# Autodesk Inventor assembly: Lady Brown
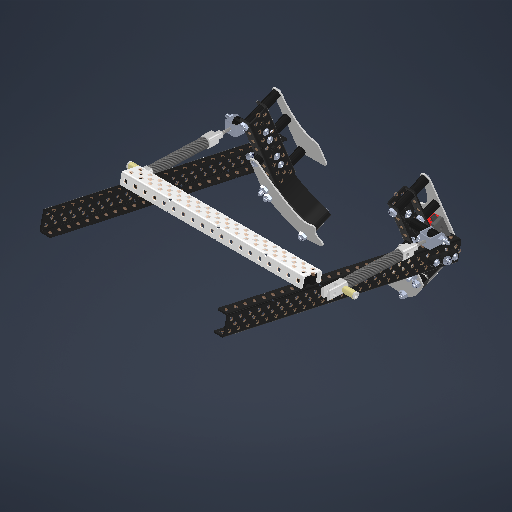
[picture p0: Inventor's stored thumbnail of the model, 512x512]
Saved by Autodesk Inventor 2025 (Build 290162000, 162)
## iProperties
Created: 2024-12-19
Part Number: Lady Brown
Document SubType Name: Assembly
Designer: Juan
Author: Juan
## Documents named in this file (33)
- C:\Users\Juan\Documents\GitHub\ATUM-VRC-High-Stakes-CAD\Robot\Subassemblies\Lady Brown.iam
- C:\Users\Juan\Documents\GitHub\ATUM-VRC-High-Stakes-CAD\VEX-CAD-Inventor\Structure\C Channel\Aluminum 1x2x1\Alu C 1x2x1x25.ipt
- C:\Users\Juan\Documents\GitHub\ATUM-VRC-High-Stakes-CAD\VEX-CAD-Inventor\Structure\C Channel\Aluminum 1x2x1\Alu C 1x2x1x19.ipt
- C:\Users\Juan\Documents\GitHub\ATUM-VRC-High-Stakes-CAD\VEX-CAD-Inventor\Motion\Spacers\Spacer Nylon .375 OD\NSpacer .375 OD x .500.ipt
- C:\Users\Juan\Documents\GitHub\ATUM-VRC-High-Stakes-CAD\VEX-CAD-Inventor\Motion\Spacers\Spacer Nylon .375 OD.ipt
- C:\Users\Juan\Documents\GitHub\ATUM-VRC-High-Stakes-CAD\VEX-CAD-Inventor\Motion\Pneumatics\Reference Parts\Pistons\Double Acting Piston Body.ipt
- C:\Users\Juan\Documents\GitHub\ATUM-VRC-High-Stakes-CAD\VEX-CAD-Inventor\Motion\Pneumatics\Reference Parts\Pistons\Double Acting Piston Rod.ipt
- C:\Users\Juan\Documents\GitHub\ATUM-VRC-High-Stakes-CAD\VEX-CAD-Inventor\Motion\Pneumatics\Legacy - SMC Pneumatics\Fitting for Cylinders.ipt
- C:\Users\Juan\Documents\GitHub\ATUM-VRC-High-Stakes-CAD\VEX-CAD-Inventor\Motion\Shaft LS\Bearing Flat.ipt
- C:\Users\Juan\Documents\GitHub\ATUM-VRC-High-Stakes-CAD\VEX-CAD-Inventor\Structure\Hardware\Screw Steel - Star\SScrew Star Smooth .500.ipt
- C:\Users\Juan\Documents\GitHub\ATUM-VRC-High-Stakes-CAD\VEX-CAD-Inventor\Structure\Hardware\Screw Steel - Star.ipt
- C:\Users\Juan\Documents\GitHub\ATUM-VRC-High-Stakes-CAD\VEX-CAD-Inventor\Structure\C Channel\Aluminum 1x3x1\Alu C 1x3x1x11.ipt
- C:\Users\Juan\Documents\GitHub\ATUM-VRC-High-Stakes-CAD\VEX-CAD-Inventor\Motion\1-Post Bearing Flat Hex Retainer.ipt
- C:\Users\Juan\Documents\GitHub\ATUM-VRC-High-Stakes-CAD\VEX-CAD-Inventor\Motion\Pneumatics\Legacy - SMC Pneumatics\Cylinder Mount.ipt
- C:\Users\Juan\Documents\GitHub\ATUM-VRC-High-Stakes-CAD\VEX-CAD-Inventor\Motion\Spacers\Spacer Nylon .375 OD\NSpacer .375 OD x .375.ipt
- C:\Users\Juan\Documents\GitHub\ATUM-VRC-High-Stakes-CAD\VEX-CAD-Inventor\Structure\Hardware\Screw Steel - Star\SScrew Star Smooth 2.250.ipt
- C:\Users\Juan\Documents\GitHub\ATUM-VRC-High-Stakes-CAD\VEX-CAD-Inventor\Structure\Hardware\Nut Nylock.ipt
- C:\Users\Juan\Documents\GitHub\ATUM-VRC-High-Stakes-CAD\VEX-CAD-Inventor\Structure\Hardware\Screw Steel - Star\SScrew Star Smooth 1.750.ipt
- C:\Users\Juan\Documents\GitHub\ATUM-VRC-High-Stakes-CAD\VEX-CAD-Inventor\Structure\Hardware\Nut Thin Nylock.ipt
- C:\Users\Juan\Documents\GitHub\ATUM-VRC-High-Stakes-CAD\VEX-CAD-Inventor\Structure\Hardware\Screw Steel - Star\SScrew Star Smooth .375.ipt
- C:\Users\Juan\Documents\GitHub\ATUM-VRC-High-Stakes-CAD\VEX-CAD-Inventor\Motion\Spacers\Spacer Nylon .375 OD\NSpacer .375 OD x .250.ipt
- C:\Users\Juan\Documents\GitHub\ATUM-VRC-High-Stakes-CAD\Protobot\Lady Brown Tabs.ipt
- C:\Users\Juan\Documents\GitHub\ATUM-VRC-High-Stakes-CAD\Protobot\Lady Brown Tab Top.ipt
- C:\Users\Juan\Documents\GitHub\ATUM-VRC-High-Stakes-CAD\VEX-CAD-Inventor\Structure\C Channel\Aluminum 1x2x1\Alu C 1x2x1x8.ipt
- C:\Users\Juan\Documents\GitHub\ATUM-VRC-High-Stakes-CAD\VEX-CAD-Inventor\Electronics\Sensors\Line Tracker - V2.ipt
- C:\Users\Juan\Documents\GitHub\ATUM-VRC-High-Stakes-CAD\Protobot\Lady Brown Ring Stop.ipt
- C:\Users\Juan\Documents\GitHub\ATUM-VRC-High-Stakes-CAD\VEX-CAD-Inventor\Motion\Spacers\Washer Steel\SWasher .375 OD x .062500.ipt
- C:\Users\Juan\Documents\GitHub\ATUM-VRC-High-Stakes-CAD\VEX-CAD-Inventor\Motion\Spacers\Washer Steel.ipt
- C:\Users\Juan\Documents\GitHub\ATUM-VRC-High-Stakes-CAD\VEX-CAD-Inventor\Structure\Hardware\Screw Steel - Star\SScrew Star Smooth 1.500.ipt
- C:\Users\Juan\Documents\GitHub\ATUM-VRC-High-Stakes-CAD\VEX-CAD-Inventor\Structure\Hardware\Screw Steel - Star\SScrew Star Smooth 2.000.ipt
- C:\Users\Juan\Documents\GitHub\ATUM-VRC-High-Stakes-CAD\VEX-CAD-Inventor\Structure\Hardware\Screw Steel - Star\SScrew Star Smooth 2.500.ipt
- C:\Users\Juan\Documents\GitHub\ATUM-VRC-High-Stakes-CAD\VEX-CAD-Inventor\Structure\Hardware\Screw Steel - Star\SScrew Star Smooth 1.250.ipt
- C:\Users\Juan\Documents\GitHub\ATUM-VRC-High-Stakes-CAD\VEX-CAD-Inventor\Structure\Hardware\Screw Steel - Star\SScrew Star Smooth .625.ipt
## Components (118 placed, 29 different names)
1. Alu C 1x2x1x25:1
2. Alu C 1x2x1x25:2
3. Alu C 1x2x1x19:1
4. NSpacer .375 OD x .500:1
5. NSpacer .375 OD x .500:2
6. Double Acting Piston Body:1
7. Double Acting Piston Rod:1
8. Fitting for Cylinders:1
9. Bearing Flat:1
10. SScrew Star Smooth .500:1
11. SScrew Star Smooth .500:2
12. Alu C 1x3x1x11:1
13. 1-Post Bearing Flat Hex Retainer:1
14. 1-Post Bearing Flat Hex Retainer:2 — Mate:77
15. Cylinder Mount:1
16. NSpacer .375 OD x .375:3 — Mate:78
17. NSpacer .375 OD x .500:4 — Mate:79
18. NSpacer .375 OD x .375:5
19. NSpacer .375 OD x .500:6
20. SScrew Star Smooth 2.250:3
21. Nut Nylock:1
22. SScrew Star Smooth 1.750:4
23. Nut Thin Nylock:1
24. Nut Nylock:2
25. SScrew Star Smooth .375:5
26. SScrew Star Smooth .375:6
27. Nut Nylock:3
28. Double Acting Piston Body:2
29. Double Acting Piston Rod:2
30. NSpacer .375 OD x .500:13
31. NSpacer .375 OD x .375:14
32. Nut Thin Nylock:4
33. Nut Thin Nylock:3
34. Nut Thin Nylock:6
35. Nut Thin Nylock:5
36. SScrew Star Smooth 2.250:12
37. NSpacer .375 OD x .500:12
38. Fitting for Cylinders:2
39. Bearing Flat:2
40. SScrew Star Smooth .500:7
41. SScrew Star Smooth .500:8
42. Alu C 1x3x1x11:2
43. NSpacer .375 OD x .500:10
44. NSpacer .375 OD x .500:11
45. Cylinder Mount:2
46. NSpacer .375 OD x .500:7
47. Nut Nylock:4
48. Nut Thin Nylock:2
49. Nut Nylock:5
50. SScrew Star Smooth .375:9
51. SScrew Star Smooth .375:10
52. Nut Nylock:6
53. 1-Post Bearing Flat Hex Retainer:3 — Mate:93
54. 1-Post Bearing Flat Hex Retainer:4 — Mate:94
55. SScrew Star Smooth 1.750:11
56. NSpacer .375 OD x .500:8 — Mate:95
57. NSpacer .375 OD x .375:9
58. NSpacer .375 OD x .375:15 — Rigid:36, Rigid:41
59. NSpacer .375 OD x .375:16 — Rigid:36, Mate:73, Mate:75, Mate:76
60. NSpacer .375 OD x .250:17 — Mate:70, Mate:72, Rigid:42
61. NSpacer .375 OD x .250:18 — Mate:71, Rigid:43
62. Lady Brown Tabs:2 — Mate:70, Mate:71, Mate:72, Mate:88, Rigid:54, Rigid:56, Rigid:67, Rigid:68, Rigid:78, Rigid:83
63. Lady Brown Tab Top:1 — Mate:73, Mate:75, Mate:76, Mate:83, Rigid:72, Rigid:76, Rigid:79
64. NSpacer .375 OD x .375:21 — Rigid:40
65. NSpacer .375 OD x .375:22 — Mate:83
66. Alu C 1x2x1x8:1 — Mate:77, Mate:78, Mate:79, Rigid:40, Rigid:41, Rigid:42, Rigid:43, Flush:1, Mate:84, Mate:85, Rigid:45, Mate:86, Mate:87, Rigid:71, Rigid:74, Rigid:81, Rigid:84
67. Line Tracker - V2:2 — Flush:1, Mate:84, Mate:85
68. NSpacer .375 OD x .375:23 — Rigid:45
69. NSpacer .375 OD x .375:24
70. Lady Brown Ring Stop:1 — Mate:86, Mate:87, Mate:88, Rigid:62, Rigid:63
71. Lady Brown Ring Stop:2 — Mate:97, Mate:98, Mate:102, Rigid:64, Rotational:3
72. Lady Brown Tabs:3 — Mate:92, Mate:96, Mate:102, Rigid:53, Rigid:55, Rigid:65, Rigid:66, Rigid:77, Rotational:5
73. NSpacer .375 OD x .250:25 — Rigid:46
74. NSpacer .375 OD x .250:26 — Mate:92, Rigid:47, Mate:96
75. Lady Brown Tab Top:2 — Mate:99, Mate:100, Mate:101, Rigid:73, Rigid:75, Rigid:80
76. Alu C 1x2x1x8:2 — Mate:93, Mate:94, Mate:95, Rigid:46, Rigid:47, Mate:97, Mate:98, Mate:99, Mate:100, Rigid:51, Rigid:52, Rotational:2, Rigid:61, Rotational:4, Rigid:82, Rigid:85
77. NSpacer .375 OD x .375:27 — Rigid:51
78. NSpacer .375 OD x .375:28
79. NSpacer .375 OD x .375:29 — Rigid:52
80. NSpacer .375 OD x .375:30 — Mate:101
81. NSpacer .375 OD x .375:31 — Rotational:2
82. NSpacer .375 OD x .375:32
83. NSpacer .375 OD x .250:33 — Rigid:54, Rigid:57
84. NSpacer .375 OD x .250:34 — Rigid:53, Rigid:60
85. NSpacer .375 OD x .250:35 — Rigid:56, Rigid:58
86. NSpacer .375 OD x .250:36 — Rigid:55, Rigid:59
87. SWasher .375 OD x .062500:1 — Rigid:58
88. SWasher .375 OD x .062500:2 — Rigid:57
89. SWasher .375 OD x .062500:3 — Rigid:60
90. SWasher .375 OD x .062500:4 — Rigid:59
91. NSpacer .375 OD x .375:37 — Rigid:61, Rigid:69
92. SScrew Star Smooth 1.500:13 — Rotational:3
93. SScrew Star Smooth 1.500:14 — Rigid:64
94. SScrew Star Smooth 1.500:15 — Rigid:63
95. SScrew Star Smooth 1.500:16 — Rigid:62
96. Nut Thin Nylock:7 — Rigid:65
97. Nut Thin Nylock:8 — Rigid:66
98. Nut Thin Nylock:9 — Rigid:68
99. Nut Thin Nylock:10 — Rigid:67
100. NSpacer .375 OD x .500:38 — Rigid:69
101. NSpacer .375 OD x .375:39 — Rigid:71
102. NSpacer .375 OD x .500:40
103. SScrew Star Smooth 2.000:17 — Rigid:72
104. SScrew Star Smooth 2.000:18 — Rigid:73
105. Nut Thin Nylock:11 — Rigid:74
106. Nut Thin Nylock:12 — Rotational:4
107. SScrew Star Smooth 2.500:20 — Rigid:75
108. SScrew Star Smooth 2.500:21 — Rigid:76
109. Nut Thin Nylock:13 — Rigid:78
110. Nut Thin Nylock:14 — Rigid:77
111. SScrew Star Smooth 1.250:22 — Rigid:80
112. SScrew Star Smooth 1.250:23 — Rigid:79
113. Nut Thin Nylock:15 — Rigid:82
114. Nut Thin Nylock:16 — Rigid:81
115. SScrew Star Smooth .625:24 — Rotational:5
116. SScrew Star Smooth .625:25 — Rigid:83
117. Nut Thin Nylock:17 — Rigid:85
118. Nut Thin Nylock:18 — Rigid:84
## Relationships (171: Mate 83, WeldJoint 80, RevoluteJoint 5, CylindricalJoint 2, Flush 1)
- [Mate]: Alu C 1x2x1x25:1 ↔ Alu C 1x2x1x19:1
- [Mate]: Alu C 1x2x1x25:1 ↔ Alu C 1x2x1x19:1
- [Mate]: Alu C 1x2x1x25:2 ↔ Alu C 1x2x1x19:1
- [Mate]: Alu C 1x2x1x25:2 ↔ Alu C 1x2x1x19:1
- [Mate]: Alu C 1x2x1x19:1 ↔ NSpacer .375 OD x .500:1
- [Mate]: Alu C 1x2x1x19:1 ↔ NSpacer .375 OD x .500:2
- [Mate]: Alu C 1x2x1x19:1 ↔ NSpacer .375 OD x .500:2
- [Mate]: Alu C 1x2x1x19:1 ↔ NSpacer .375 OD x .500:1
- [Mate]: Alu C 1x2x1x25:1 ↔ NSpacer .375 OD x .500:2
- [Mate]: Double Acting Piston Body:1 ↔ Double Acting Piston Rod:1
- [CylindricalJoint]: Double Acting Piston Body:1 ↔ Double Acting Piston Rod:1
- [Mate]: Double Acting Piston Body:1 ↔ Fitting for Cylinders:1
- [Mate]: Double Acting Piston Body:1 ↔ Fitting for Cylinders:1
- [Mate]: Alu C 1x2x1x25:1 ↔ Bearing Flat:1
- [Mate]: Alu C 1x2x1x25:1 ↔ Bearing Flat:1
- [Mate]: Alu C 1x2x1x25:1 ↔ Bearing Flat:1
- [WeldJoint]: Bearing Flat:1 ↔ SScrew Star Smooth .500:2
- [WeldJoint]: Bearing Flat:1 ↔ SScrew Star Smooth .500:1
- [Mate]: Alu C 1x3x1x11:1 ↔ 1-Post Bearing Flat Hex Retainer:2
- [Mate]: Alu C 1x3x1x11:1 ↔ 1-Post Bearing Flat Hex Retainer:2
- [Mate]: Alu C 1x3x1x11:1 ↔ 1-Post Bearing Flat Hex Retainer:1
- [Mate]: Alu C 1x3x1x11:1 ↔ 1-Post Bearing Flat Hex Retainer:1
- [Mate]: Alu C 1x3x1x11:1 ↔ 1-Post Bearing Flat Hex Retainer:2
- [Mate]: Alu C 1x3x1x11:1 ↔ 1-Post Bearing Flat Hex Retainer:1
- [Mate]: Bearing Flat:1 ↔ 1-Post Bearing Flat Hex Retainer:2
- [Mate]: Double Acting Piston Rod:1 ↔ Cylinder Mount:1
- [Mate]: 1-Post Bearing Flat Hex Retainer:1 ↔ Cylinder Mount:1
- [WeldJoint]: NSpacer .375 OD x .500:4 ↔ NSpacer .375 OD x .375:5
- [Mate]: Cylinder Mount:1 ↔ NSpacer .375 OD x .500:6
- [Mate]: Cylinder Mount:1 ↔ NSpacer .375 OD x .500:6
- [WeldJoint]: Alu C 1x3x1x11:1 ↔ SScrew Star Smooth 2.250:3
- [WeldJoint]: Cylinder Mount:1 ↔ Nut Nylock:1
- [WeldJoint]: Alu C 1x3x1x11:1 ↔ SScrew Star Smooth 1.750:4
- [WeldJoint]: Bearing Flat:1 ↔ Nut Thin Nylock:1
- [WeldJoint]: Alu C 1x3x1x11:1 ↔ SScrew Star Smooth .375:6
- [WeldJoint]: Alu C 1x3x1x11:1 ↔ SScrew Star Smooth .375:5
- [WeldJoint]: 1-Post Bearing Flat Hex Retainer:1 ↔ Nut Nylock:2
- [WeldJoint]: 1-Post Bearing Flat Hex Retainer:2 ↔ Nut Nylock:3
- [Mate]: Double Acting Piston Body:2 ↔ Double Acting Piston Rod:2
- [Mate]: Double Acting Piston Body:2 ↔ Fitting for Cylinders:2
- [Mate]: Double Acting Piston Body:2 ↔ Fitting for Cylinders:2
- [Mate]: Double Acting Piston Rod:2 ↔ Cylinder Mount:2
- [Mate]: Cylinder Mount:2 ↔ NSpacer .375 OD x .500:7
- [CylindricalJoint]: Double Acting Piston Body:2 ↔ Double Acting Piston Rod:2
- [WeldJoint]: Bearing Flat:2 ↔ SScrew Star Smooth .500:7
- [WeldJoint]: Bearing Flat:2 ↔ SScrew Star Smooth .500:8
- [WeldJoint]: Cylinder Mount:2 ↔ Nut Nylock:4
- [WeldJoint]: Bearing Flat:2 ↔ Nut Thin Nylock:2
- [WeldJoint]: Alu C 1x3x1x11:2 ↔ SScrew Star Smooth .375:9
- [WeldJoint]: Alu C 1x3x1x11:2 ↔ SScrew Star Smooth .375:10
- [Mate]: Alu C 1x3x1x11:2 ↔ 1-Post Bearing Flat Hex Retainer:3
- [Mate]: Alu C 1x3x1x11:2 ↔ 1-Post Bearing Flat Hex Retainer:3
- [Mate]: Alu C 1x3x1x11:2 ↔ 1-Post Bearing Flat Hex Retainer:3
- [Mate]: Alu C 1x3x1x11:2 ↔ 1-Post Bearing Flat Hex Retainer:4
- [Mate]: Alu C 1x3x1x11:2 ↔ 1-Post Bearing Flat Hex Retainer:4
- [Mate]: Alu C 1x3x1x11:2 ↔ 1-Post Bearing Flat Hex Retainer:4
- [WeldJoint]: Alu C 1x3x1x11:2 ↔ SScrew Star Smooth 1.750:11
- [Mate]: Alu C 1x2x1x25:2 ↔ Bearing Flat:2
- [Mate]: Alu C 1x2x1x25:2 ↔ Bearing Flat:2
- [Mate]: Alu C 1x2x1x25:2 ↔ Bearing Flat:2
- [Mate]: Bearing Flat:2 ↔ SScrew Star Smooth 1.750:11
- [Mate]: Cylinder Mount:2 ↔ NSpacer .375 OD x .500:7
- [WeldJoint]: Nut Nylock:5 ↔ 1-Post Bearing Flat Hex Retainer:3
- [WeldJoint]: Nut Nylock:6 ↔ 1-Post Bearing Flat Hex Retainer:4
- [WeldJoint]: NSpacer .375 OD x .500:8 ↔ NSpacer .375 OD x .375:9
- [Mate]: Alu C 1x2x1x25:2 ↔ Double Acting Piston Body:2
- [Mate] (0.7937 mm): Alu C 1x2x1x25:2 ↔ Double Acting Piston Body:2
- [Mate]: Alu C 1x3x1x11:1 ↔ Alu C 1x3x1x11:2
- [Mate]: Alu C 1x3x1x11:1 ↔ Alu C 1x3x1x11:2
- [RevoluteJoint] (0.7937 mm): Alu C 1x2x1x25:1 ↔ Double Acting Piston Body:1
- [WeldJoint] (6.35 mm): Double Acting Piston Rod:1 ↔ Cylinder Mount:1
- [WeldJoint] (6.35 mm): Double Acting Piston Rod:2 ↔ Cylinder Mount:2
- [Mate]: Cylinder Mount:2 ↔ NSpacer .375 OD x .375:9
- [Mate]: 1-Post Bearing Flat Hex Retainer:2 ↔ NSpacer .375 OD x .375:3
- [WeldJoint]: Cylinder Mount:1 ↔ NSpacer .375 OD x .375:5
- [Mate]: Alu C 1x2x1x25:2 ↔ NSpacer .375 OD x .500:11
- [Mate]: Alu C 1x2x1x25:2 ↔ NSpacer .375 OD x .500:10
- [Mate]: Alu C 1x2x1x25:2 ↔ NSpacer .375 OD x .500:10
- [Mate]: Alu C 1x2x1x25:2 ↔ NSpacer .375 OD x .500:11
- [WeldJoint]: Alu C 1x2x1x25:1 ↔ NSpacer .375 OD x .500:12
- [WeldJoint]: NSpacer .375 OD x .375:3 ↔ NSpacer .375 OD x .500:12
- [WeldJoint]: NSpacer .375 OD x .500:13 ↔ NSpacer .375 OD x .375:14
- [Mate]: NSpacer .375 OD x .500:13 ↔ SScrew Star Smooth 1.750:11
- [Mate]: Alu C 1x2x1x25:2 ↔ NSpacer .375 OD x .500:13
- [Mate]: NSpacer .375 OD x .375:14 ↔ 1-Post Bearing Flat Hex Retainer:4
- [WeldJoint]: Alu C 1x2x1x25:1 ↔ Nut Thin Nylock:4
- [WeldJoint]: Alu C 1x2x1x25:1 ↔ Nut Thin Nylock:3
- [WeldJoint]: SScrew Star Smooth 2.250:12 ↔ Alu C 1x3x1x11:2
- [WeldJoint]: Alu C 1x2x1x25:2 ↔ Nut Thin Nylock:6
- [WeldJoint]: Alu C 1x2x1x25:2 ↔ Nut Thin Nylock:5
- [Mate]: SScrew Star Smooth 2.250:12 ↔ Nut Nylock:4
- [Mate]: SScrew Star Smooth 2.250:12 ↔ NSpacer .375 OD x .375:9
- Rigid:36 [WeldJoint]: NSpacer .375 OD x .375:15 ↔ NSpacer .375 OD x .375:16
- Mate:70: NSpacer .375 OD x .250:17 ↔ Lady Brown Tabs:2
- Mate:71: NSpacer .375 OD x .250:18 ↔ Lady Brown Tabs:2
- Mate:72: NSpacer .375 OD x .250:17 ↔ Lady Brown Tabs:2
- Mate:73: NSpacer .375 OD x .375:16 ↔ Lady Brown Tab Top:1
- Mate:75: NSpacer .375 OD x .375:16 ↔ Lady Brown Tab Top:1
- Mate:76: NSpacer .375 OD x .375:16 ↔ Lady Brown Tab Top:1
- [WeldJoint]: NSpacer .375 OD x .375:21 ↔ NSpacer .375 OD x .375:22
- Mate:77: 1-Post Bearing Flat Hex Retainer:2 ↔ Alu C 1x2x1x8:1
- Mate:78: NSpacer .375 OD x .375:3 ↔ Alu C 1x2x1x8:1
- Mate:79: NSpacer .375 OD x .500:4 ↔ Alu C 1x2x1x8:1
- Rigid:40 [WeldJoint]: NSpacer .375 OD x .375:21 ↔ Alu C 1x2x1x8:1
- Rigid:41 [WeldJoint]: NSpacer .375 OD x .375:15 ↔ Alu C 1x2x1x8:1
- Rigid:42 [WeldJoint]: NSpacer .375 OD x .250:17 ↔ Alu C 1x2x1x8:1
- Rigid:43 [WeldJoint]: NSpacer .375 OD x .250:18 ↔ Alu C 1x2x1x8:1
- Mate:83: Lady Brown Tab Top:1 ↔ NSpacer .375 OD x .375:22
- Flush:1 (-6.35 mm): Alu C 1x2x1x8:1 ↔ Line Tracker - V2:2
- Mate:84: Alu C 1x2x1x8:1 ↔ Line Tracker - V2:2
- Mate:85: Alu C 1x2x1x8:1 ↔ Line Tracker - V2:2
- [WeldJoint]: NSpacer .375 OD x .375:23 ↔ NSpacer .375 OD x .375:24
- Rigid:45 [WeldJoint]: Alu C 1x2x1x8:1 ↔ NSpacer .375 OD x .375:23
- Mate:86: Alu C 1x2x1x8:1 ↔ Lady Brown Ring Stop:1
- Mate:87: Alu C 1x2x1x8:1 ↔ Lady Brown Ring Stop:1
- Mate:88: Lady Brown Tabs:2 ↔ Lady Brown Ring Stop:1
- Mate:92: Lady Brown Tabs:3 ↔ NSpacer .375 OD x .250:26
- Mate:93: 1-Post Bearing Flat Hex Retainer:3 ↔ Alu C 1x2x1x8:2
- Mate:94: 1-Post Bearing Flat Hex Retainer:4 ↔ Alu C 1x2x1x8:2
- Mate:95: NSpacer .375 OD x .500:8 ↔ Alu C 1x2x1x8:2
- Rigid:46 [WeldJoint]: NSpacer .375 OD x .250:25 ↔ Alu C 1x2x1x8:2
- Rigid:47 [WeldJoint]: NSpacer .375 OD x .250:26 ↔ Alu C 1x2x1x8:2
- Mate:96: Lady Brown Tabs:3 ↔ NSpacer .375 OD x .250:26
- Mate:97: Lady Brown Ring Stop:2 ↔ Alu C 1x2x1x8:2
- Mate:98: Lady Brown Ring Stop:2 ↔ Alu C 1x2x1x8:2
- Mate:99: Lady Brown Tab Top:2 ↔ Alu C 1x2x1x8:2
- Mate:100: Lady Brown Tab Top:2 ↔ Alu C 1x2x1x8:2
- [WeldJoint]: NSpacer .375 OD x .375:27 ↔ NSpacer .375 OD x .375:28
- [WeldJoint]: NSpacer .375 OD x .375:29 ↔ NSpacer .375 OD x .375:30
- [WeldJoint]: NSpacer .375 OD x .375:31 ↔ NSpacer .375 OD x .375:32
- Rigid:51 [WeldJoint]: Alu C 1x2x1x8:2 ↔ NSpacer .375 OD x .375:27
- Rigid:52 [WeldJoint]: Alu C 1x2x1x8:2 ↔ NSpacer .375 OD x .375:29
- Rotational:2 [RevoluteJoint]: Alu C 1x2x1x8:2 ↔ NSpacer .375 OD x .375:31
- Mate:101: Lady Brown Tab Top:2 ↔ NSpacer .375 OD x .375:30
- Mate:102: Lady Brown Ring Stop:2 ↔ Lady Brown Tabs:3
- Rigid:53 [WeldJoint]: Lady Brown Tabs:3 ↔ NSpacer .375 OD x .250:34
- Rigid:54 [WeldJoint]: Lady Brown Tabs:2 ↔ NSpacer .375 OD x .250:33
- Rigid:55 [WeldJoint]: Lady Brown Tabs:3 ↔ NSpacer .375 OD x .250:36
- Rigid:56 [WeldJoint]: Lady Brown Tabs:2 ↔ NSpacer .375 OD x .250:35
- Rigid:57 [WeldJoint]: NSpacer .375 OD x .250:33 ↔ SWasher .375 OD x .062500:2
- Rigid:58 [WeldJoint]: NSpacer .375 OD x .250:35 ↔ SWasher .375 OD x .062500:1
- Rigid:59 [WeldJoint]: NSpacer .375 OD x .250:36 ↔ SWasher .375 OD x .062500:4
- Rigid:60 [WeldJoint]: NSpacer .375 OD x .250:34 ↔ SWasher .375 OD x .062500:3
- Rigid:61 [WeldJoint]: Alu C 1x2x1x8:2 ↔ NSpacer .375 OD x .375:37
- Rigid:62 [WeldJoint]: Lady Brown Ring Stop:1 ↔ SScrew Star Smooth 1.500:16
- Rigid:63 [WeldJoint]: Lady Brown Ring Stop:1 ↔ SScrew Star Smooth 1.500:15
- Rigid:64 [WeldJoint]: Lady Brown Ring Stop:2 ↔ SScrew Star Smooth 1.500:14
- Rotational:3 [RevoluteJoint]: Lady Brown Ring Stop:2 ↔ SScrew Star Smooth 1.500:13
- Rigid:65 [WeldJoint]: Lady Brown Tabs:3 ↔ Nut Thin Nylock:7
- Rigid:66 [WeldJoint]: Lady Brown Tabs:3 ↔ Nut Thin Nylock:8
- Rigid:67 [WeldJoint]: Lady Brown Tabs:2 ↔ Nut Thin Nylock:10
- Rigid:68 [WeldJoint]: Lady Brown Tabs:2 ↔ Nut Thin Nylock:9
- Rigid:69 [WeldJoint]: NSpacer .375 OD x .375:37 ↔ NSpacer .375 OD x .500:38
- [WeldJoint]: NSpacer .375 OD x .375:39 ↔ NSpacer .375 OD x .500:40
- Rigid:71 [WeldJoint]: Alu C 1x2x1x8:1 ↔ NSpacer .375 OD x .375:39
- Rigid:72 [WeldJoint]: Lady Brown Tab Top:1 ↔ SScrew Star Smooth 2.000:17
- Rigid:73 [WeldJoint]: Lady Brown Tab Top:2 ↔ SScrew Star Smooth 2.000:18
- Rigid:74 [WeldJoint]: Alu C 1x2x1x8:1 ↔ Nut Thin Nylock:11
- Rotational:4 [RevoluteJoint]: Alu C 1x2x1x8:2 ↔ Nut Thin Nylock:12
- Rigid:75 [WeldJoint]: Lady Brown Tab Top:2 ↔ SScrew Star Smooth 2.500:20
- Rigid:76 [WeldJoint]: Lady Brown Tab Top:1 ↔ SScrew Star Smooth 2.500:21
- Rigid:77 [WeldJoint]: Lady Brown Tabs:3 ↔ Nut Thin Nylock:14
- Rigid:78 [WeldJoint]: Lady Brown Tabs:2 ↔ Nut Thin Nylock:13
- Rigid:79 [WeldJoint]: Lady Brown Tab Top:1 ↔ SScrew Star Smooth 1.250:23
- Rigid:80 [WeldJoint]: Lady Brown Tab Top:2 ↔ SScrew Star Smooth 1.250:22
- Rigid:81 [WeldJoint]: Alu C 1x2x1x8:1 ↔ Nut Thin Nylock:16
- Rigid:82 [WeldJoint]: Alu C 1x2x1x8:2 ↔ Nut Thin Nylock:15
- Rotational:5 [RevoluteJoint]: Lady Brown Tabs:3 ↔ SScrew Star Smooth .625:24
- Rigid:83 [WeldJoint]: Lady Brown Tabs:2 ↔ SScrew Star Smooth .625:25
- Rigid:84 [WeldJoint]: Alu C 1x2x1x8:1 ↔ Nut Thin Nylock:18
- Rigid:85 [WeldJoint]: Alu C 1x2x1x8:2 ↔ Nut Thin Nylock:17
## Named parameters: d1821_d1818 = 0 mm, d1789_d1094 = 0 mm, d1790_d1097 = 0 mm, d1791_d1068_d1063 = 0 mm, d1792_d1069_d1064 = 0 deg, d1793_d1070_d1065 = -19.05 mm, d1794_d1071_d1066 = -19.09226 mm, d1795_d1072_d1067 = -69.85 mm, d131_d126_d116 = 0 mm, d152_d116 = 0 mm, d173_d116 = 0 mm, d174_d116 = 0 mm, d175_d116 = 0 mm, d201_d200 = 0 mm
